# Autodesk Inventor assembly: Montagem_suporte_termopar
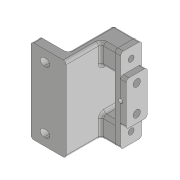
[picture p0: Inventor's stored thumbnail of the model, 180x180]
Saved by Autodesk Inventor 2020 (Build 240168000, 168)
## iProperties
Created: 2022-07-21
Part Number: Montagem_suporte_termopar
Document SubType Name: Assembly
Designer: gabri
Author: gabri
## Documents named in this file (4)
- C:\Users\gabri\OneDrive\Área de Trabalho\Calorimetro 2022\Inventor\Montagem_suporte_termopar.iam
- C:\Users\gabri\OneDrive\Área de Trabalho\Calorimetro 2022\Inventor\suporte_termopar.ipt
- C:\Users\gabri\OneDrive\Área de Trabalho\Calorimetro 2022\Inventor\suporte_termopar_al.ipt
- C:\Users\gabri\OneDrive\Área de Trabalho\Calorimetro 2022\Inventor\tampa_suporte_termopar.ipt
## Components (3 placed, 3 different names)
1. suporte_termopar:1 — Alinhamento:1, Alinhamento:2
2. suporte_termopar_al:1 — Alinhamento:1, Alinhamento:2, Alinhamento:3, Alinhamento:4
3. tampa_suporte_termopar:1 — Alinhamento:3, Alinhamento:4
## Relationships (4: Flush 4)
- Alinhamento:1 [Flush]: suporte_termopar:1 ↔ suporte_termopar_al:1
- Alinhamento:2 [Flush]: suporte_termopar:1 ↔ suporte_termopar_al:1
- Alinhamento:3 [Flush]: suporte_termopar_al:1 ↔ tampa_suporte_termopar:1
- Alinhamento:4 [Flush]: suporte_termopar_al:1 ↔ tampa_suporte_termopar:1
